# Autodesk Inventor assembly: LegBaseSlashCutCrankUnit
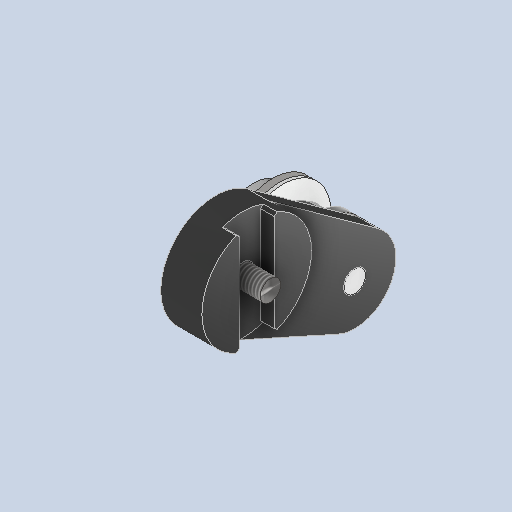
[picture p0: Inventor's stored thumbnail of the model, 512x512]
Saved by Autodesk Inventor 2024.2 (Build 282272000, 272)
## iProperties
Created: 2024-01-06
Part Number: LegBaseSlashCutCrankUnit
Document SubType Name: Assembly
Designer: Masato Kubotera
Author: Masato Kubotera
## Documents named in this file (8)
- C:\Users\masato\OneDrive - Chiba Institute of Technology\CIT Brains\RoboCup2024\Mechanic\SUSTAINA-OP2\NativeFiles\Boby\LowerLimb\Legs\LegBases\LegBaseSlashCutCrankUnit.iam
- C:\Users\masato\OneDrive - Chiba Institute of Technology\CIT Brains\RoboCup2024\Mechanic\SUSTAINA-OP2\NativeFiles\Boby\COTS\Bushes\LED-0606.ipt
- C:\Users\masato\OneDrive - Chiba Institute of Technology\CIT Brains\RoboCup2024\Mechanic\SUSTAINA-OP2\NativeFiles\Boby\COTS\Washers\Metal\UUW-0412-10H.ipt
- C:\Users\masato\OneDrive - Chiba Institute of Technology\CIT Brains\RoboCup2024\Mechanic\SUSTAINA-OP2\NativeFiles\Boby\COTS\Screws\ScrewsWithShoulder\DBTSY4-8-4-DHC-PC.ipt
- C:\Users\masato\OneDrive - Chiba Institute of Technology\CIT Brains\RoboCup2024\Mechanic\SUSTAINA-OP2\NativeFiles\Boby\CommonDesignedComponents\SlashCutLongCrankFrame.ipt
- C:\Users\masato\OneDrive - Chiba Institute of Technology\CIT Brains\RoboCup2024\Mechanic\SUSTAINA-OP2\NativeFiles\Boby\COTS\Washers\Resin\TT-0614-05.ipt
- C:\Users\masato\OneDrive - Chiba Institute of Technology\CIT Brains\RoboCup2024\Mechanic\SUSTAINA-OP2\NativeFiles\Boby\COTS\Washers\Metal\UUW-0614-10H.ipt
- C:\Users\masato\OneDrive - Chiba Institute of Technology\CIT Brains\RoboCup2024\Mechanic\SUSTAINA-OP2\NativeFiles\Boby\COTS\Screws\LowHeadCapScrew\ULC-0308.ipt
## Components (7 placed, 7 different names)
1. SlashCutLongCrankFrame:1 — Mate:1, Flush:3, Flush:1, Insert:1, Insert:3
2. LED-0606:1 — Insert:2, Angle:1
3. ULC-0308:1 — Insert:3
4. UUW-0412-10H:1 — Insert:1, Insert:2, Insert:6
5. TT-0614-05:1 — Insert:4
6. UUW-0614-10H:1 — Insert:4, Insert:5
7. DBTSY4-8-4-DHC-PC:1 — Insert:5, Insert:6
## Relationships (10: Insert 6, Flush 2, Mate 1, Angle 1)
- Mate:1: SlashCutLongCrankFrame:1
- Flush:3: SlashCutLongCrankFrame:1
- Flush:1 (20.25 mm): SlashCutLongCrankFrame:1
- Insert:1: SlashCutLongCrankFrame:1 ↔ UUW-0412-10H:1
- Insert:2: LED-0606:1 ↔ UUW-0412-10H:1
- Angle:1 (0 deg): LED-0606:1
- Insert:3: SlashCutLongCrankFrame:1 ↔ ULC-0308:1
- Insert:4: TT-0614-05:1 ↔ UUW-0614-10H:1
- Insert:5: UUW-0614-10H:1 ↔ DBTSY4-8-4-DHC-PC:1
- Insert:6: UUW-0412-10H:1 ↔ DBTSY4-8-4-DHC-PC:1
